# Autodesk Inventor assembly: ___Verkettung
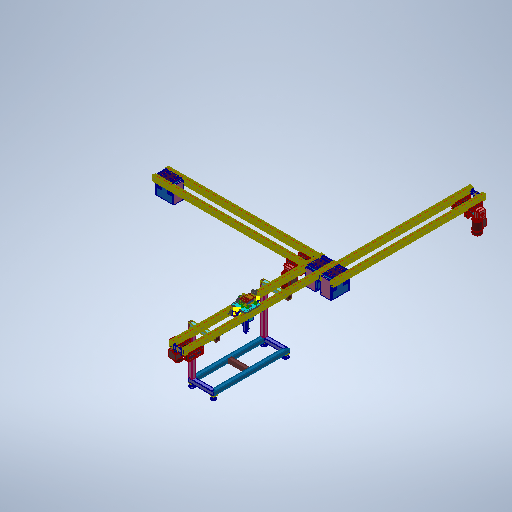
[picture p0: Inventor's stored thumbnail of the model, 512x512]
Saved by Autodesk Inventor 2025.1 (Build 291241000, 241)
## iProperties
Created: 2023-11-17
Part Number: ___Verkettung
Material: Generisch
Document SubType Name: Assembly
Designer: RP
Source: Unknown
Title: Gurtband WT-240
Author: RP
Revision Number: ANY
## iProperties of the stored document MemberDocs/xAaaaaqdaAaaaaaaaAaaaqgxrLh
Created: 2023-11-17
Part Number: ___Verkettung
Material: Generisch
Document SubType Name: Assembly
Designer: RP
Source: Unknown
Title: Gurtband WT-240
Author: RP
Revision Number: ANY
## Documents named in this file (29)
- C:\Users\Erik\Erik\Hochschule\3. Semester\CAD\CAD-Paspa\Useless Box\__Projekt_Useless_Box.iam
- C:\Users\Erik\Erik\Hochschule\3. Semester\CAD\Useless Box\_Verkettung\_VK_Hub-Station.iam
- C:\Users\Erik\Erik\Hochschule\3. Semester\CAD\Useless Box\_Verkettung\__VK_Transferband.iam
- C:\Users\Erik\Erik\Hochschule\3. Semester\CAD\Useless Box\_Verkettung\__VK_Gestell.iam
- C:\Users\Erik\Erik\Hochschule\3. Semester\CAD\Useless Box\_Verkettung\__VK_WT_beladen.iam
- C:\Users\Erik\Erik\Hochschule\3. Semester\CAD\Useless Box\_Verkettung\__VK_Sensor_Palette_1_0.ipt
- C:\Users\Erik\Erik\Hochschule\3. Semester\CAD\Useless Box\Eigene Bauteile\ER_Positionierungseinheit_Backe_int.ipt
- C:\Users\Erik\Erik\Hochschule\3. Semester\CAD\Useless Box\Eigene Bauteile\JH_Positionierungseinheit_Vertikalbegrenzung_int.ipt
- C:\Users\Erik\Erik\Hochschule\3. Semester\CAD\Useless Box\Eigene Bauteile\TS_Positionierungseinheit_Rahmen_int.iam
- C:\Users\Erik\Documents\Inventor\Content Center Files\R2025\en-US\ISO 4762(2)\ISO 4762 - M8 x 40ISO.ipt
- C:\Users\Erik\Documents\Inventor\Content Center Files\R2025\en-US\ISO 2338(2)\ISO 2338 - 6 m6 x 50.ipt
- C:\Users\Erik\Erik\Hochschule\3. Semester\CAD\Useless Box\Eigene Bauteile\ER_Positionierungseinheit_Backe_int_MIR.ipt
- C:\Users\Erik\Documents\Inventor\Content Center Files\R2025\en-US\ISO 4026\ISO 4026 - M8 x 40 - ISO.ipt
- C:\Users\Erik\Erik\Hochschule\3. Semester\CAD\Useless Box\Eigene Bauteile\ER_Positionierungseinheit_Backe_int_MIR1.ipt
- C:\Users\Erik\Erik\Hochschule\3. Semester\CAD\CAD-Paspa\Useless Box\_Verkettung\_VK_Hub-Station.iam
- C:\Users\Erik\Erik\Hochschule\3. Semester\CAD\CAD-Paspa\Useless Box\_Verkettung\__VK_Transferband.iam
- C:\Users\Erik\Erik\Hochschule\3. Semester\CAD\CAD-Paspa\Useless Box\_Verkettung\__VK_Gestell.iam
- C:\Users\Erik\Erik\Hochschule\3. Semester\CAD\CAD-Paspa\Useless Box\_Verkettung\__VK_WT_beladen.iam
- C:\Users\Erik\Erik\Hochschule\3. Semester\CAD\CAD-Paspa\Useless Box\_Verkettung\__VK_Sensor_Palette_1_0.ipt
- C:\Users\Erik\Erik\Hochschule\3. Semester\CAD\CAD-Paspa\Useless Box\Eigene Bauteile\ER_Positionierungseinheit_Backe_int.ipt
- C:\Users\Erik\Erik\Hochschule\3. Semester\CAD\CAD-Paspa\Useless Box\Eigene Bauteile\JH_Positionierungseinheit_Vertikalbegrenzung_int.ipt
- C:\Users\Erik\Erik\Hochschule\3. Semester\CAD\CAD-Paspa\Useless Box\Eigene Bauteile\TS_Positionierungseinheit_Rahmen_int.iam
- C:\Users\Erik\Erik\Hochschule\3. Semester\CAD\CAD-Paspa\Useless Box\Standart Bauteile\ISO 4762 - M6 x 12ISO.ipt
- C:\Users\Erik\Erik\Hochschule\3. Semester\CAD\CAD-Paspa\Useless Box\Standart Bauteile\ISO 4026 - M6 x 16 - ISO.ipt
- C:\Users\Erik\Erik\Hochschule\3. Semester\CAD\CAD-Paspa\Useless Box\Standart Bauteile\ISO 4762 - M8 x 40ISO.ipt
- C:\Users\Erik\Erik\Hochschule\3. Semester\CAD\CAD-Paspa\Useless Box\Standart Bauteile\ISO 2338 - 6 m6 x 50.ipt
- C:\Users\Erik\Erik\Hochschule\3. Semester\CAD\CAD-Paspa\Useless Box\Standart Bauteile\ISO 4026 - M8 x 40 - ISO.ipt
- C:\Users\Erik\Erik\Hochschule\3. Semester\CAD\CAD-Paspa\Useless Box\Kaufteile\Rexroth_Profil_40x40_168mm\Rexroth_Profil_40x40_168mm.ipt
- C:\Users\Erik\Erik\Hochschule\3. Semester\CAD\Useless Box\__Projekt_Useless_Box.iam
## Components (33 placed, 13 different names)
1. __VK_Transferband:1 [sub-assembly] — Mate:107, Passend:108, Fluchtend:96, Passend:109, Passend:110, Fluchtend:98, Passend:112, Fluchtend:99, Passend:113, Fluchtend:100, Fluchtend:101, Mate:123
2. __VK_Sensor_Palette_1_0:1 — Passend:109, Passend:110
3. _VK_Hub-Station:1 [sub-assembly] — Fluchtend:84, Passend:101, Flush:102, Mate:124
4. __VK_WT_beladen:6 [sub-assembly] — Fluchtend:67, Passend:95, Passend:101, Flush:104
5. __VK_Gestell:2 [sub-assembly] — Passend:108, Fluchtend:96, Flush:102
6. __VK_Transferband:2 [sub-assembly] — Fluchtend:98, Passend:112, Fluchtend:99
7. __VK_Transferband:3 [sub-assembly] — Passend:113, Fluchtend:100, Fluchtend:101
8. ER_Positionierungseinheit_Backe_int:3 — Mate:126, Mate:127, Mate:128
9. ISO 4762 M8 x 40:3 — Mate:129, Mate:130
10. ISO 2338 6 m6 x 50:5 — Mate:132, Flush:107
11. ISO 4026 M8 x 40:5 — Mate:131, Flush:106
12. ISO 2338 6 m6 x 50:6
13. ISO 4026 M8 x 40:6
14. ER_Positionierungseinheit_Backe_int_MIR1:1
15. ISO 4762 M8 x 40:4
16. ISO 2338 6 m6 x 50:7
17. ISO 4026 M8 x 40:7
18. ISO 2338 6 m6 x 50:8
19. ISO 4026 M8 x 40:8
20. ER_Positionierungseinheit_Backe_int_MIR:1
21. ISO 4762 M8 x 40:2
22. ISO 2338 6 m6 x 50:3
23. ISO 2338 6 m6 x 50:4
24. ISO 4026 M8 x 40:3
25. ISO 4026 M8 x 40:4
26. JH_Positionierungseinheit_Vertikalbegrenzung_int:1
27. TS_Positionierungseinheit_Rahmen_int:1 [sub-assembly] — Mate:117, Mate:118, Mate:119, Mate:120, Mate:121, Mate:122, Flush:103, Mate:123, Mate:124, Flush:104, Mate:125, Flush:105, Mate:126, Mate:127, Mate:128, Mate:129, Mate:130, Mate:131, Flush:106, Mate:132, Flush:107
28. ISO 2338 6 m6 x 50:1 — Mate:122, Flush:103
29. ISO 4762 M8 x 40:1 — Mate:120, Mate:121
30. ER_Positionierungseinheit_Backe_int:2 — Mate:117, Mate:118, Mate:119
31. ISO 2338 6 m6 x 50:2
32. ISO 4026 M8 x 40:1 — Mate:125, Flush:105
33. ISO 4026 M8 x 40:2
## Relationships (43: Mate 27, Flush 16)
- [Mate]: __VK_Transferband:1
- [Mate]: __VK_Transferband:1
- [Flush]: __VK_Transferband:1
- [Mate]: __VK_Transferband:1
- Fluchtend:67 [Flush]: __VK_WT_beladen:6
- [Flush]: _VK_Hub-Station:1
- Fluchtend:84 [Flush]: _VK_Hub-Station:1
- [Flush]: __VK_Transferband:1
- Passend:95 [Mate]: __VK_WT_beladen:6
- Passend:101 [Mate]: _VK_Hub-Station:1 ↔ __VK_WT_beladen:6
- Mate:107: __VK_Transferband:1
- Passend:108 [Mate]: __VK_Transferband:1 ↔ __VK_Gestell:2
- Fluchtend:96 [Flush]: __VK_Transferband:1 ↔ __VK_Gestell:2
- Passend:109 [Mate]: __VK_Transferband:1 ↔ __VK_Sensor_Palette_1_0:1
- Passend:110 [Mate]: __VK_Transferband:1 ↔ __VK_Sensor_Palette_1_0:1
- Fluchtend:98 [Flush]: __VK_Transferband:1 ↔ __VK_Transferband:2
- Passend:112 [Mate]: __VK_Transferband:1 ↔ __VK_Transferband:2
- Fluchtend:99 [Flush]: __VK_Transferband:1 ↔ __VK_Transferband:2
- Passend:113 [Mate]: __VK_Transferband:1 ↔ __VK_Transferband:3
- Fluchtend:100 [Flush]: __VK_Transferband:1 ↔ __VK_Transferband:3
- Fluchtend:101 [Flush]: __VK_Transferband:1 ↔ __VK_Transferband:3
- Flush:102 (-541.5 mm): _VK_Hub-Station:1 ↔ __VK_Gestell:2
- Mate:117: TS_Positionierungseinheit_Rahmen_int:1 ↔ ER_Positionierungseinheit_Backe_int:2
- Mate:118: TS_Positionierungseinheit_Rahmen_int:1 ↔ ER_Positionierungseinheit_Backe_int:2
- Mate:119: TS_Positionierungseinheit_Rahmen_int:1 ↔ ER_Positionierungseinheit_Backe_int:2
- Mate:120: TS_Positionierungseinheit_Rahmen_int:1 ↔ ISO 4762 M8 x 40:1
- Mate:121: TS_Positionierungseinheit_Rahmen_int:1 ↔ ISO 4762 M8 x 40:1
- Mate:122: TS_Positionierungseinheit_Rahmen_int:1 ↔ ISO 2338 6 m6 x 50:1
- Flush:103: TS_Positionierungseinheit_Rahmen_int:1 ↔ ISO 2338 6 m6 x 50:1
- Mate:123 (101.5 mm): __VK_Transferband:1 ↔ TS_Positionierungseinheit_Rahmen_int:1
- Mate:124: _VK_Hub-Station:1 ↔ TS_Positionierungseinheit_Rahmen_int:1
- Flush:104: __VK_WT_beladen:6 ↔ TS_Positionierungseinheit_Rahmen_int:1
- Mate:125: TS_Positionierungseinheit_Rahmen_int:1 ↔ ISO 4026 M8 x 40:1
- Flush:105: TS_Positionierungseinheit_Rahmen_int:1 ↔ ISO 4026 M8 x 40:1
- Mate:126: ER_Positionierungseinheit_Backe_int:3 ↔ TS_Positionierungseinheit_Rahmen_int:1
- Mate:127: ER_Positionierungseinheit_Backe_int:3 ↔ TS_Positionierungseinheit_Rahmen_int:1
- Mate:128: ER_Positionierungseinheit_Backe_int:3 ↔ TS_Positionierungseinheit_Rahmen_int:1
- Mate:129: ISO 4762 M8 x 40:3 ↔ TS_Positionierungseinheit_Rahmen_int:1
- Mate:130: ISO 4762 M8 x 40:3 ↔ TS_Positionierungseinheit_Rahmen_int:1
- Mate:131: ISO 4026 M8 x 40:5 ↔ TS_Positionierungseinheit_Rahmen_int:1
- Flush:106: ISO 4026 M8 x 40:5 ↔ TS_Positionierungseinheit_Rahmen_int:1
- Mate:132: ISO 2338 6 m6 x 50:5 ↔ TS_Positionierungseinheit_Rahmen_int:1
- Flush:107: ISO 2338 6 m6 x 50:5 ↔ TS_Positionierungseinheit_Rahmen_int:1
